# Autodesk Inventor assembly: CL3-100
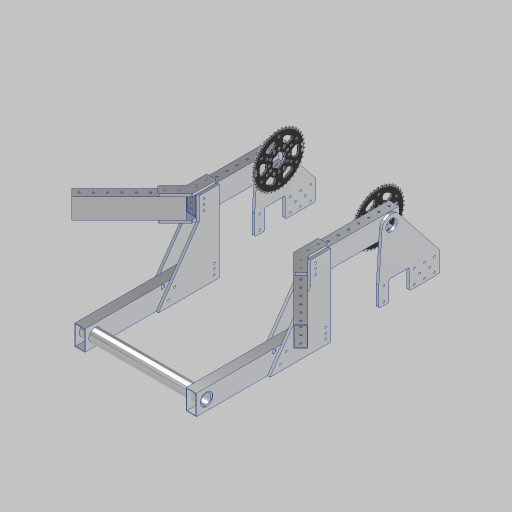
[picture p0: Inventor's stored thumbnail of the model, 512x512]
Saved by Autodesk Inventor 2023.5 (Build 275446000, 446)
## iProperties
Created: 2025-01-28
Part Number: CL3-100
Document SubType Name: Assembly
Designer: slick
Mass: 5241.21 g
Surface Area: 12801.1 cm^2
Volume: 1941.19 cm^3
Density: 2.7 g/cm^3
Author: slick
## Documents named in this file (12)
- C:\Users\slick\OneDrive\Desktop\2025-ReefScape---CAD\Climber\CL3\CL3-100.iam
- C:\Users\slick\OneDrive\Desktop\2025-ReefScape---CAD\Climber\CL3\CL3-001.ipt
- C:\Users\slick\OneDrive\Desktop\2025-ReefScape---CAD\Climber\CL3\CL3-002.ipt
- C:\Users\slick\OneDrive\Desktop\2025-ReefScape---CAD\Climber\CL3\CL3-003.ipt
- C:\Users\slick\OneDrive\Desktop\2025-ReefScape---CAD\Climber\CL3\CL3-004.ipt
- C:\Users\slick\OneDrive\Desktop\2025-ReefScape---CAD\Climber\CL3\CL3-006.ipt
- C:\Users\slick\OneDrive\Desktop\2025-ReefScape---CAD\Field Items\Full Field\FE-2025\GE-25201.iam
- C:\Users\slick\OneDrive\Desktop\2025-ReefScape---CAD\Climber\CL3\CL3-007.ipt
- C:\Users\slick\OneDrive\Desktop\2025-ReefScape---CAD\Climber\CL3\CL3-009.ipt
- C:\Users\slick\OneDrive\Desktop\2025-ReefScape---CAD\Elevator\EL2\EL2-005.ipt
- C:\Users\slick\OneDrive\Desktop\2025-ReefScape---CAD\Climber\CL3\CL3-010.ipt
- C:\Users\slick\OneDrive\Desktop\2025-ReefScape---CAD\COMMON PARTS\SPROCKETS\35\42t 35 Chain Spline XL Plate SprocketWCP-0984.ipt
## Components (23 placed, 11 different names)
1. CL3-001:1 — Mate:9, Flush:5, Mate:11, Mate:16, Symmetry:1, Angle:1, Flush:24, Insert:5, Insert:6, Insert:7, Insert:10, Angle:2, Insert:11, Insert:12, Insert:13, Insert:14, Mate:38
2. CL3-002:1 — Flush:24, Insert:3, Insert:4, Insert:8
3. CL3-003:1 — Insert:26, Insert:27
4. CL3-001:2 — Mate:9, Flush:5, Mate:14, Symmetry:1, Flush:25, Mate:36, Mate:40, Insert:18, Insert:19, Insert:20, Insert:21, Insert:24, Insert:25
5. CL3-002:2 — Flush:25, Insert:22, Insert:23
6. CL3-003:2 — Mate:29, Flush:26, Flush:27, Mate:33, Mate:34, Insert:15, Angle:3, Insert:16, Insert:17
7. CL3-004:3 — Mate:11, Mate:16, Angle:1, Flush:28
8. CL3-004:4 — Mate:14, Flush:28, Mate:36
9. CL3-006:1 — Tangent:1, Mate:21, Mate:33, Mate:34
10. GE-25201:1 [sub-assembly] — Mate:20, Tangent:1, Mate:21
11. CL3-007:1 — Mate:29, Flush:26, Flush:27
12. CL3-009:1 — Insert:3, Insert:4, Insert:5, Insert:6
13. CL3-009:2 — Insert:7, Insert:8
14. EL2-005:2 — Insert:10, Angle:2
15. CL3-010:1 — Insert:11, Insert:12
16. CL3-010:2 — Insert:13, Insert:14, Insert:16, Insert:17
17. EL2-005:3 — Insert:15, Angle:3
18. 42t 35 Chain Spline XL Plate SprocketWCP-0984:1 — Mate:38
19. 42t 35 Chain Spline XL Plate SprocketWCP-0984:2 — Mate:40
20. CL3-009:3 — Insert:18, Insert:19
21. CL3-009:4 — Insert:20, Insert:21, Insert:22, Insert:23
22. CL3-010:3 — Insert:25
23. CL3-010:4 — Insert:24, Insert:26, Insert:27
## Relationships (47: Insert 24, Mate 12, Flush 6, Angle 3, Symmetry 1, Tangent 1)
- Mate:9 (254 mm): CL3-001:1 ↔ CL3-001:2
- Flush:5: CL3-001:1 ↔ CL3-001:2
- Mate:11: CL3-001:1 ↔ CL3-004:3
- Mate:14: CL3-001:2 ↔ CL3-004:4
- Mate:16: CL3-001:1 ↔ CL3-004:3
- Symmetry:1: CL3-001:1 ↔ CL3-001:2
- Mate:20: GE-25201:1
- Tangent:1: CL3-006:1 ↔ GE-25201:1
- Mate:21 (-76.2 mm): CL3-006:1 ↔ GE-25201:1
- Angle:1 (90 deg): CL3-001:1 ↔ CL3-004:3
- Flush:24: CL3-001:1 ↔ CL3-002:1
- Flush:25: CL3-001:2 ↔ CL3-002:2
- Mate:29: CL3-003:2 ↔ CL3-007:1
- Flush:26: CL3-003:2 ↔ CL3-007:1
- Flush:27: CL3-003:2 ↔ CL3-007:1
- Insert:3: CL3-002:1 ↔ CL3-009:1
- Insert:4: CL3-002:1 ↔ CL3-009:1
- Insert:5: CL3-001:1 ↔ CL3-009:1
- Insert:6: CL3-001:1 ↔ CL3-009:1
- Insert:7: CL3-001:1 ↔ CL3-009:2
- Insert:8: CL3-002:1 ↔ CL3-009:2
- Mate:33: CL3-003:2 ↔ CL3-006:1
- Mate:34: CL3-003:2 ↔ CL3-006:1
- Insert:10: CL3-001:1 ↔ EL2-005:2
- Angle:2 (0 deg): CL3-001:1 ↔ EL2-005:2
- Insert:11: CL3-001:1 ↔ CL3-010:1
- Insert:12: CL3-001:1 ↔ CL3-010:1
- Insert:13: CL3-001:1 ↔ CL3-010:2
- Insert:14: CL3-001:1 ↔ CL3-010:2
- Insert:15: CL3-003:2 ↔ EL2-005:3
- Angle:3 (0 deg): CL3-003:2 ↔ EL2-005:3
- Insert:16: CL3-003:2 ↔ CL3-010:2
- Insert:17: CL3-003:2 ↔ CL3-010:2
- Flush:28: CL3-004:3 ↔ CL3-004:4
- Mate:36: CL3-001:2 ↔ CL3-004:4
- Mate:38: CL3-001:1 ↔ 42t 35 Chain Spline XL Plate SprocketWCP-0984:1
- Mate:40: CL3-001:2 ↔ 42t 35 Chain Spline XL Plate SprocketWCP-0984:2
- Insert:18: CL3-001:2 ↔ CL3-009:3
- Insert:19: CL3-001:2 ↔ CL3-009:3
- Insert:20: CL3-001:2 ↔ CL3-009:4
- Insert:21: CL3-001:2 ↔ CL3-009:4
- Insert:22: CL3-002:2 ↔ CL3-009:4
- Insert:23: CL3-002:2 ↔ CL3-009:4
- Insert:24: CL3-001:2 ↔ CL3-010:4
- Insert:25: CL3-001:2 ↔ CL3-010:3
- Insert:26: CL3-003:1 ↔ CL3-010:4
- Insert:27: CL3-003:1 ↔ CL3-010:4
